# Autodesk Inventor assembly: DriveSideAssembly
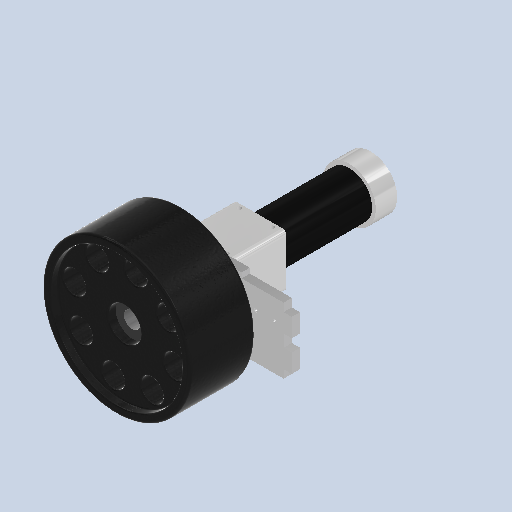
[picture p0: Inventor's stored thumbnail of the model, 512x512]
Saved by Autodesk Inventor 2022 (Build 260153000, 153)
## iProperties
Created: 2021-05-22
Part Number: DriveSideAssembly
Document SubType Name: Assembly
Designer: M3rob
Mass: 10195.5 g
Surface Area: 4709.21 cm^2
Volume: 4918.96 cm^3
Density: 2.07269 g/cm^3
Author: M3rob
## Documents named in this file (6)
- C:\Users\M3rob\Documents\GrabCAD\FireBird 250 Pound Gaming Machine\Drafts\FrameDrafts\Draft_04\Assemblies\DriveSideAssembly.iam
- C:\Users\M3rob\Documents\GrabCAD\FireBird 250 Pound Gaming Machine\Drafts\FrameDrafts\Draft_04\Chassis and Mounting\DriveSideFrame_03.ipt
- C:\Users\M3rob\Documents\GrabCAD\FireBird 250 Pound Gaming Machine\Drafts\FrameDrafts\Draft_04\Drive\GearboxMockup.ipt
- C:\Users\M3rob\Documents\GrabCAD\FireBird 250 Pound Gaming Machine\Drafts\FrameDrafts\Draft_04\Electronics\MagMotorMockup.ipt
- C:\Users\M3rob\Documents\GrabCAD\FireBird 250 Pound Gaming Machine\Drafts\FrameDrafts\Draft_04\Hardware\91251A583_Bolts-WeaponSprocket.ipt
- C:\Users\M3rob\Documents\GrabCAD\FireBird 250 Pound Gaming Machine\Drafts\FrameDrafts\Draft_04\Assemblies\DriveWheelCastingAssembly.iam
## Components (8 placed, 5 different names)
1. DriveSideFrame_03:1 — Mate:1, Mate:2, Mate:3, Mate:4, Mate:5, Mate:6, Mate:7, Mate:8, Mate:9, Mate:10, Mate:11
2. GearboxMockup:1 — Mate:1, Mate:2, Mate:3, Mate:12, Mate:13, Mate:14, Angle:1, Mate:15
3. MagMotorMockup:1 — Mate:12, Mate:13
4. 91251A583_Bolts-WeaponSprocket:1 — Mate:4, Mate:10
5. 91251A583_Bolts-WeaponSprocket:2 — Mate:6, Mate:11
6. 91251A583_Bolts-WeaponSprocket:3 — Mate:7, Mate:9
7. 91251A583_Bolts-WeaponSprocket:4 — Mate:5, Mate:8
8. DriveWheelCastingAssembly:1 [sub-assembly] — Mate:14, Angle:1, Mate:15
## Relationships (16: Mate 15, Angle 1)
- Mate:1: DriveSideFrame_03:1 ↔ GearboxMockup:1
- Mate:2: DriveSideFrame_03:1 ↔ GearboxMockup:1
- Mate:3: DriveSideFrame_03:1 ↔ GearboxMockup:1
- Mate:4: DriveSideFrame_03:1 ↔ 91251A583_Bolts-WeaponSprocket:1
- Mate:5: DriveSideFrame_03:1 ↔ 91251A583_Bolts-WeaponSprocket:4
- Mate:6: DriveSideFrame_03:1 ↔ 91251A583_Bolts-WeaponSprocket:2
- Mate:7: DriveSideFrame_03:1 ↔ 91251A583_Bolts-WeaponSprocket:3
- Mate:8: DriveSideFrame_03:1 ↔ 91251A583_Bolts-WeaponSprocket:4
- Mate:9: DriveSideFrame_03:1 ↔ 91251A583_Bolts-WeaponSprocket:3
- Mate:10: DriveSideFrame_03:1 ↔ 91251A583_Bolts-WeaponSprocket:1
- Mate:11: DriveSideFrame_03:1 ↔ 91251A583_Bolts-WeaponSprocket:2
- Mate:12: GearboxMockup:1 ↔ MagMotorMockup:1
- Mate:13: GearboxMockup:1 ↔ MagMotorMockup:1
- Mate:14: GearboxMockup:1 ↔ DriveWheelCastingAssembly:1
- Angle:1 (0 deg): GearboxMockup:1 ↔ DriveWheelCastingAssembly:1
- Mate:15 (12.7 mm): GearboxMockup:1 ↔ DriveWheelCastingAssembly:1
